# Autodesk Inventor assembly: VersaPlanetary Input MiniCIM
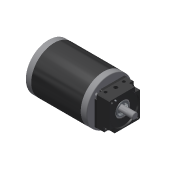
[picture p0: Inventor's stored thumbnail of the model, 180x180]
Saved by Autodesk Inventor 2013 (Build 170138000, 138)
## iProperties
Created: 2013-12-15
Part Number: VersaPlanetary Input MiniCIM
Document SubType Name: Assembly
Designer: Nemo
Author: Nemo
## Documents named in this file (9)
- H:\Nemo\Documents\Robotics\COTS Parts\VersaPlanetary\VersaPlanetary Input MiniCIM.iam
- H:\Nemo\Documents\Robotics\COTS Parts\VersaPlanetary\Components\VersaPlanetary Case Motor Side.ipt
- H:\Nemo\Documents\Robotics\COTS Parts\VersaPlanetary\Components\VersaPlanetary Shaft Holder.ipt
- H:\Nemo\Documents\Robotics\COTS Parts\Bearings - VexPro\Radial Bearing - 17mm x 26mm x 5mm.ipt
- H:\Nemo\Documents\Robotics\COTS Parts\VersaPlanetary\Components\VersaPlanetary RS550 shaft piece.ipt
- H:\Nemo\Documents\Robotics\COTS Parts\VersaPlanetary\Components\VersaPlanetary shaft holder clip ring.ipt
- H:\Nemo\Documents\Robotics\COTS Parts\VersaPlanetary\Components\VersaPlanetary pin.ipt
- H:\Nemo\Documents\Robotics\COTS Parts\VersaPlanetary\Components\VersaPlanetary Mount Plate - BAG.ipt
- H:\Nemo\Documents\Robotics\COTS Parts\Motors\Mini CIM.ipt
## Components (8 placed, 8 different names)
1. VersaPlanetary Case Motor Side:1 — Mate:1, Mate:2, Insert:5, Mate:6, Flush:2, Flush:3, Mate:11, Flush:4, Flush:5
2. VersaPlanetary Shaft Holder:1 — Mate:3, Mate:4, Mate:5, Flush:1, Insert:4
3. Radial Bearing - 17mm x 26mm x 5mm:1 — Mate:1, Mate:2, Mate:3, Mate:4
4. VersaPlanetary RS550 shaft piece:1 — Mate:5, Flush:1
5. VersaPlanetary shaft holder clip ring:1 — Insert:4
6. VersaPlanetary pin:1 — Insert:5
7. VersaPlanetary Mount Plate - BAG:1 — Mate:6, Flush:2, Flush:3, Insert:6
8. Mini CIM:1 — Insert:6
## Relationships (15: Mate 7, Flush 5, Insert 3)
- Mate:1: VersaPlanetary Case Motor Side:1 ↔ Radial Bearing - 17mm x 26mm x 5mm:1
- Mate:2: VersaPlanetary Case Motor Side:1 ↔ Radial Bearing - 17mm x 26mm x 5mm:1
- Mate:3: VersaPlanetary Shaft Holder:1 ↔ Radial Bearing - 17mm x 26mm x 5mm:1
- Mate:4: VersaPlanetary Shaft Holder:1 ↔ Radial Bearing - 17mm x 26mm x 5mm:1
- Mate:5: VersaPlanetary Shaft Holder:1 ↔ VersaPlanetary RS550 shaft piece:1
- Flush:1: VersaPlanetary Shaft Holder:1 ↔ VersaPlanetary RS550 shaft piece:1
- Insert:4: VersaPlanetary Shaft Holder:1 ↔ VersaPlanetary shaft holder clip ring:1
- Insert:5: VersaPlanetary Case Motor Side:1 ↔ VersaPlanetary pin:1
- Mate:6: VersaPlanetary Case Motor Side:1 ↔ VersaPlanetary Mount Plate - BAG:1
- Flush:2: VersaPlanetary Case Motor Side:1 ↔ VersaPlanetary Mount Plate - BAG:1
- Flush:3: VersaPlanetary Case Motor Side:1 ↔ VersaPlanetary Mount Plate - BAG:1
- Mate:11: VersaPlanetary Case Motor Side:1
- Flush:4: VersaPlanetary Case Motor Side:1
- Flush:5: VersaPlanetary Case Motor Side:1
- Insert:6: VersaPlanetary Mount Plate - BAG:1 ↔ Mini CIM:1
